# Autodesk Inventor assembly: A_MiniDrone
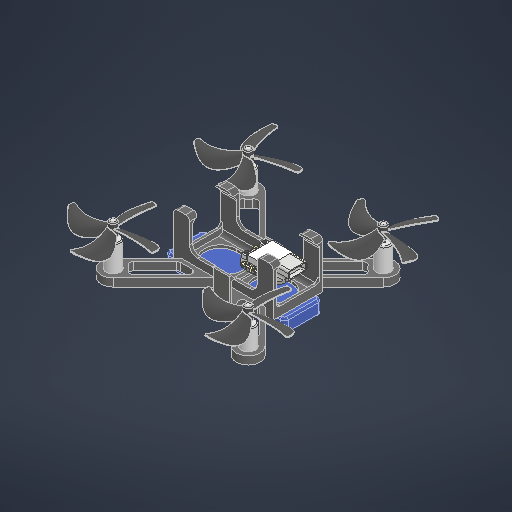
[picture p0: Inventor's stored thumbnail of the model, 512x512]
Saved by Autodesk Inventor 2026.2 (Build 302298000, 298)
## iProperties
Created: 2026-02-08
Part Number: A_MiniDrone
Document SubType Name: Assembly
Designer: FAL
Author: FAL
## Documents named in this file (7)
- C:\Users\FAL\git\ESP32-Drone\Hardware\CAD\V3\A_MiniDrone.iam
- C:\Users\FAL\git\ESP32-Drone\Hardware\CAD\V3\P_Motor.ipt
- C:\Users\FAL\git\ESP32-Drone\Hardware\CAD\V3\P_DroneCase.ipt
- C:\Users\FAL\projects\_libary\electronic\microcontroller\esp32\esp32-C3\ESP32-C3_SEEED\ESP32-C3_SEEED\ESP32-C3_SEEED.ipt
- C:\Users\FAL\git\ESP32-Drone\Hardware\CAD\V3\P_Akku_1S.ipt
- C:\Users\FAL\git\ESP32-Drone\Hardware\CAD\V3\P_Prop_4_blade.ipt
- C:\Users\FAL\git\ESP32-Drone\Hardware\CAD\V3\P_Halter.ipt
## Components (12 placed, 6 different names)
1. P_Motor:1 — Passend:3, Passend:10, Fluchtend:7
2. P_Motor:2 — Passend:1, Passend:12, Fluchtend:5
3. P_Motor:3 — Passend:2, Passend:9, Fluchtend:4
4. P_Motor:4 — Passend:4, Passend:11, Fluchtend:6
5. P_DroneCase:1 — Fluchtend:1, Fluchtend:2, Fluchtend:3, Passend:1, Passend:2, Passend:3, Passend:4, Passend:13, Passend:16
6. ESP32-C3_SEEED:1 — Passend:8
7. P_Akku_1S:1 — Passend:6, Passend:13
8. P_Prop_4_blade:1 — Passend:9, Fluchtend:4
9. P_Prop_4_blade:2 — Passend:12, Fluchtend:5
10. P_Prop_4_blade:3 — Passend:10, Fluchtend:7
11. P_Prop_4_blade:4 — Passend:11, Fluchtend:6
12. P_Halter:1 — Passend:14, Passend:15, Passend:16
## Relationships (21: Mate 14, Flush 7)
- Fluchtend:1 [Flush]: P_DroneCase:1
- Fluchtend:2 [Flush]: P_DroneCase:1
- Fluchtend:3 [Flush]: P_DroneCase:1
- Passend:1 [Mate]: P_Motor:2 ↔ P_DroneCase:1
- Passend:2 [Mate]: P_Motor:3 ↔ P_DroneCase:1
- Passend:3 [Mate]: P_Motor:1 ↔ P_DroneCase:1
- Passend:4 [Mate]: P_Motor:4 ↔ P_DroneCase:1
- Passend:6 [Mate]: P_Akku_1S:1
- Passend:8 [Mate]: ESP32-C3_SEEED:1
- Passend:9 [Mate]: P_Motor:3 ↔ P_Prop_4_blade:1
- Fluchtend:4 [Flush]: P_Motor:3 ↔ P_Prop_4_blade:1
- Passend:10 [Mate]: P_Motor:1 ↔ P_Prop_4_blade:3
- Passend:11 [Mate]: P_Motor:4 ↔ P_Prop_4_blade:4
- Passend:12 [Mate]: P_Motor:2 ↔ P_Prop_4_blade:2
- Fluchtend:5 [Flush]: P_Motor:2 ↔ P_Prop_4_blade:2
- Fluchtend:6 [Flush]: P_Motor:4 ↔ P_Prop_4_blade:4
- Fluchtend:7 [Flush]: P_Motor:1 ↔ P_Prop_4_blade:3
- Passend:13 [Mate]: P_DroneCase:1 ↔ P_Akku_1S:1
- Passend:14 [Mate]: P_Halter:1
- Passend:15 [Mate]: P_Halter:1
- Passend:16 [Mate]: P_DroneCase:1 ↔ P_Halter:1
